# Autodesk Inventor assembly: HyperCube Evolution - Single Z motor 1.0
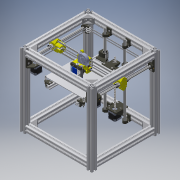
[picture p0: Inventor's stored thumbnail of the model, 180x180]
Saved by Autodesk Inventor 2016 (Build 200138000, 138)
## iProperties
Created: 2017-04-13
Part Number: HyperCube Evolution - Single Z motor 1.0
Document SubType Name: Assembly
Designer: Scott
Author: Scott
## Documents named in this file (16)
- E:\Scott Projects\3D Printing\CoreXY\HyperCube Evolution - Single Z motor 1.0.iam
- E:\Scott Projects\3D Printing\CoreXY\HyperCube Evolution.iam
- E:\Scott Projects\3D Printing\CoreXY\Z Axis Liner Rail Bracket Assembly - Left 1.0.iam
- E:\Scott Projects\3D Printing\CoreXY\Z Axis Liner Rail Bracket Assembly - Right 1.0.iam
- E:\Scott Projects\3D Printing\CoreXY\Linear rail - Z.ipt
- E:\Scott Projects\3D Printing\CoreXY\X Axis Assembly 1.0.iam
- E:\Scott Projects\3D Printing\CoreXY\X Carriage Assembly.iam
- E:\Scott Projects\3D Printing\CoreXY\Build Platform Assembly 1.0.iam
- C:\Users\Scott\Documents\Inventor\Content Center Files\R2016\en-US\ANSI B18.3.4M(1)\ANSI B18.3.4M - M5 x 0.8 x 10(2).ipt
- E:\Scott Projects\3D Printing\CoreXY\Z Motor Mount 1.0.ipt
- E:\Scott Projects\3D Printing\CoreXY\Extruder Assembly.iam
- E:\Scott Projects\3D Printing\CoreXY\GT2_20T.ipt
- E:\Scott Projects\3D Printing\CoreXY\Belt 1.ipt
- E:\Scott Projects\3D Printing\CoreXY\Belt 2.ipt
- E:\Scott Projects\3D Printing\CoreXY\NEMA 17 T8x8 Assembly.iam
- C:\Users\Scott\Documents\Inventor\Content Center Files\R2016\en-US\ANSI B18.3.1M(1)\ANSI B18.3.1M - M3x0.5 x 12(2).ipt
## Components (26 placed, 15 different names)
1. HyperCube Evolution:1 [sub-assembly] — Flush:1, Flush:2, Flush:3, Mate:1, Mate:2, Mate:3, Mate:4, Mate:5, Mate:6, Mate:7, Mate:8, Mate:11, Mate:12, Mate:17, Mate:18, Mate:23, Mate:24, Mate:25, Mate:26, Mate:34, Mate:35
2. Z Axis Liner Rail Bracket Assembly - Left 1.0:1 [sub-assembly] — Mate:1, Mate:3, Insert:1, Insert:3
3. Z Axis Liner Rail Bracket Assembly - Left 1.0:2 [sub-assembly] — Mate:2, Mate:4, Mate:9
4. Z Axis Liner Rail Bracket Assembly - Right 1.0:1 [sub-assembly] — Mate:5, Mate:6, Insert:2
5. Z Axis Liner Rail Bracket Assembly - Right 1.0:2 [sub-assembly] — Mate:7, Mate:8, Mate:10
6. Linear rail - Z:1 — Insert:1, Mate:9, Mate:20
7. Linear rail - Z:2 — Insert:2, Mate:10, Mate:19
8. X Axis Assembly 1.0:1 [sub-assembly] — Mate:11, Mate:12, Mate:13, Mate:14, Flush:6, Flush:7, Mate:28, Mate:29, Mate:32, Mate:37, Mate:38
9. X Carriage Assembly:1 [sub-assembly] — Mate:13, Mate:14, Mate:22, Flush:4, Flush:5, Mate:30, Mate:31, Mate:32, Mate:39, Mate:40
10. Build Platform Assembly 1.0:1 [sub-assembly] — Mate:19, Mate:20, Mate:21
11. Broached Hexagon Socket Button Head Cap Screw - Metric M5 x 0.8 x 10:1 — Insert:3
12. Z Motor Mount 1.0:1 — Mate:17, Mate:18, Mate:42, Insert:4, Insert:5, Insert:6, Insert:7, Insert:8, Angle:1, Insert:9, Insert:10, Insert:11, Insert:12
13. Extruder Assembly:1 [sub-assembly] — Mate:22, Flush:4, Flush:5
14. GT2_20T:1 — Mate:23, Flush:7, Mate:27, Mate:33
15. GT2_20T:2 — Mate:24, Flush:6, Mate:36, Mate:41
16. Belt 1:1 — Mate:25, Mate:26, Mate:27, Mate:28, Mate:29, Mate:30, Mate:31, Mate:33
17. Belt 2:1 — Mate:34, Mate:35, Mate:36, Mate:37, Mate:38, Mate:39, Mate:40, Mate:41
18. Broached Hexagon Socket Button Head Cap Screw - Metric M5 x 0.8 x 10:2 — Insert:5
19. Broached Hexagon Socket Button Head Cap Screw - Metric M5 x 0.8 x 10:3 — Insert:7
20. Broached Hexagon Socket Button Head Cap Screw - Metric M5 x 0.8 x 10:4 — Insert:6
21. Broached Hexagon Socket Button Head Cap Screw - Metric M5 x 0.8 x 10:5 — Insert:4
22. NEMA 17 T8x8 Assembly:1 [sub-assembly] — Insert:8, Angle:1
23. Broached Socket Head Cap Screw - Metric M3x0.5 x 12:1 — Insert:12
24. Broached Socket Head Cap Screw - Metric M3x0.5 x 12:2 — Insert:11
25. Broached Socket Head Cap Screw - Metric M3x0.5 x 12:3 — Insert:10
26. Broached Socket Head Cap Screw - Metric M3x0.5 x 12:4 — Insert:9
## Relationships (60: Mate 40, Insert 12, Flush 7, Angle 1)
- Flush:1: HyperCube Evolution:1
- Flush:2: HyperCube Evolution:1
- Flush:3: HyperCube Evolution:1
- Mate:1: HyperCube Evolution:1 ↔ Z Axis Liner Rail Bracket Assembly - Left 1.0:1
- Mate:2: HyperCube Evolution:1 ↔ Z Axis Liner Rail Bracket Assembly - Left 1.0:2
- Mate:3: HyperCube Evolution:1 ↔ Z Axis Liner Rail Bracket Assembly - Left 1.0:1
- Mate:4: HyperCube Evolution:1 ↔ Z Axis Liner Rail Bracket Assembly - Left 1.0:2
- Mate:5: HyperCube Evolution:1 ↔ Z Axis Liner Rail Bracket Assembly - Right 1.0:1
- Mate:6: HyperCube Evolution:1 ↔ Z Axis Liner Rail Bracket Assembly - Right 1.0:1
- Mate:7: HyperCube Evolution:1 ↔ Z Axis Liner Rail Bracket Assembly - Right 1.0:2
- Mate:8: HyperCube Evolution:1 ↔ Z Axis Liner Rail Bracket Assembly - Right 1.0:2
- Insert:1: Z Axis Liner Rail Bracket Assembly - Left 1.0:1 ↔ Linear rail - Z:1
- Insert:2: Z Axis Liner Rail Bracket Assembly - Right 1.0:1 ↔ Linear rail - Z:2
- Mate:9: Z Axis Liner Rail Bracket Assembly - Left 1.0:2 ↔ Linear rail - Z:1
- Mate:10: Z Axis Liner Rail Bracket Assembly - Right 1.0:2 ↔ Linear rail - Z:2
- Mate:11: HyperCube Evolution:1 ↔ X Axis Assembly 1.0:1
- Mate:12: HyperCube Evolution:1 ↔ X Axis Assembly 1.0:1
- Mate:13: X Axis Assembly 1.0:1 ↔ X Carriage Assembly:1
- Mate:14: X Axis Assembly 1.0:1 ↔ X Carriage Assembly:1
- Insert:3: Z Axis Liner Rail Bracket Assembly - Left 1.0:1 ↔ Broached Hexagon Socket Button Head Cap Screw - Metric M5 x 0.8 x 10:1
- Mate:17: HyperCube Evolution:1 ↔ Z Motor Mount 1.0:1
- Mate:18: HyperCube Evolution:1 ↔ Z Motor Mount 1.0:1
- Mate:19: Linear rail - Z:2 ↔ Build Platform Assembly 1.0:1
- Mate:20: Linear rail - Z:1 ↔ Build Platform Assembly 1.0:1
- Mate:21: Build Platform Assembly 1.0:1
- Mate:22: X Carriage Assembly:1 ↔ Extruder Assembly:1
- Flush:4: X Carriage Assembly:1 ↔ Extruder Assembly:1
- Flush:5: X Carriage Assembly:1 ↔ Extruder Assembly:1
- Mate:23: HyperCube Evolution:1 ↔ GT2_20T:1
- Mate:24: HyperCube Evolution:1 ↔ GT2_20T:2
- Flush:6: X Axis Assembly 1.0:1 ↔ GT2_20T:2
- Flush:7: X Axis Assembly 1.0:1 ↔ GT2_20T:1
- Mate:25: HyperCube Evolution:1 ↔ Belt 1:1
- Mate:26: HyperCube Evolution:1 ↔ Belt 1:1
- Mate:27: GT2_20T:1 ↔ Belt 1:1
- Mate:28: X Axis Assembly 1.0:1 ↔ Belt 1:1
- Mate:29: X Axis Assembly 1.0:1 ↔ Belt 1:1
- Mate:30: X Carriage Assembly:1 ↔ Belt 1:1
- Mate:31: X Carriage Assembly:1 ↔ Belt 1:1
- Mate:32 (100 mm): X Axis Assembly 1.0:1 ↔ X Carriage Assembly:1
- Mate:33 (0.25 mm): GT2_20T:1 ↔ Belt 1:1
- Mate:34: HyperCube Evolution:1 ↔ Belt 2:1
- Mate:35: HyperCube Evolution:1 ↔ Belt 2:1
- Mate:36: GT2_20T:2 ↔ Belt 2:1
- Mate:37: X Axis Assembly 1.0:1 ↔ Belt 2:1
- Mate:38: X Axis Assembly 1.0:1 ↔ Belt 2:1
- Mate:39: X Carriage Assembly:1 ↔ Belt 2:1
- Mate:40: X Carriage Assembly:1 ↔ Belt 2:1
- Mate:41 (0.25 mm): GT2_20T:2 ↔ Belt 2:1
- Mate:42: Z Motor Mount 1.0:1
- Insert:4: Z Motor Mount 1.0:1 ↔ Broached Hexagon Socket Button Head Cap Screw - Metric M5 x 0.8 x 10:5
- Insert:5: Z Motor Mount 1.0:1 ↔ Broached Hexagon Socket Button Head Cap Screw - Metric M5 x 0.8 x 10:2
- Insert:6: Z Motor Mount 1.0:1 ↔ Broached Hexagon Socket Button Head Cap Screw - Metric M5 x 0.8 x 10:4
- Insert:7: Z Motor Mount 1.0:1 ↔ Broached Hexagon Socket Button Head Cap Screw - Metric M5 x 0.8 x 10:3
- Insert:8: Z Motor Mount 1.0:1 ↔ NEMA 17 T8x8 Assembly:1
- Angle:1 (0 deg): Z Motor Mount 1.0:1 ↔ NEMA 17 T8x8 Assembly:1
- Insert:9: Z Motor Mount 1.0:1 ↔ Broached Socket Head Cap Screw - Metric M3x0.5 x 12:4
- Insert:10: Z Motor Mount 1.0:1 ↔ Broached Socket Head Cap Screw - Metric M3x0.5 x 12:3
- Insert:11: Z Motor Mount 1.0:1 ↔ Broached Socket Head Cap Screw - Metric M3x0.5 x 12:2
- Insert:12: Z Motor Mount 1.0:1 ↔ Broached Socket Head Cap Screw - Metric M3x0.5 x 12:1
